# Autodesk Inventor assembly: Luftkissenboot
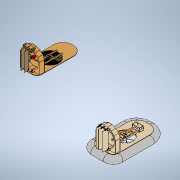
[picture p0: Inventor's stored thumbnail of the model, 180x180]
Saved by Autodesk Inventor 2020.3 (Build 243373010, 373A)
## iProperties
Company: HTBLuVA St. Pölten
Created: 2020-02-10
Part Number: Luftkissenboot
Document SubType Name: Assembly
Designer: Stefan Deimel
Mass: 445608 g
Surface Area: 116837 cm^2
Volume: 445608 cm^3
Density: 1 g/cm^3
Project: Diplomarbeit
Description: Luftkissenboot
Author: Stefan
Title: Luftkissenboot
Subject: Diplomarbeit
Revision Number: 3.1
## Documents named in this file (25)
- D:\Stefan\Schule\HTL\Diplomarbeit\git\Inventor\Luftkissenboot.iam
- D:\Stefan\Schule\HTL\Diplomarbeit\git\Inventor\Schlauchoot.ipt
- D:\Stefan\Schule\HTL\Diplomarbeit\git\Inventor\Aufbau.ipt
- D:\Stefan\Schule\HTL\Diplomarbeit\git\Inventor\Motor.ipt
- D:\Stefan\Schule\HTL\Diplomarbeit\git\Inventor\LenkungHinten.ipt
- D:\Stefan\Schule\HTL\Diplomarbeit\git\Inventor\Lenkung_hinten_verbindung.ipt
- D:\Stefan\Schule\HTL\Diplomarbeit\git\Inventor\Lenkung_vorne.ipt
- D:\Stefan\Schule\HTL\Diplomarbeit\git\Inventor\Propeller.ipt
- D:\Stefan\Schule\HTL\Diplomarbeit\git\Inventor\GitterUnten.ipt
- D:\Stefan\Schule\HTL\Diplomarbeit\git\Inventor\FahneHolz.ipt
- D:\Stefan\Schule\HTL\Diplomarbeit\git\Inventor\Fahnen_Halter v8.ipt
- D:\Stefan\Schule\HTL\Diplomarbeit\git\Inventor\Fahnen_Halter v8_1.ipt
- C:\Users\Stefan\Documents\Inventor\Content Center Files\R2020\de-DE\ANSI B18.2.4.2M\ANSI B18.2.4.2M - M5x0,8 - 8.ipt
- C:\Users\Stefan\Documents\Inventor\Content Center Files\R2020\de-DE\ISO 4016\ISO 4016 - M5 x 30.ipt
- D:\Stefan\Schule\HTL\Diplomarbeit\git\Inventor\FahenVerbindung_maybe.ipt
- D:\Stefan\Schule\HTL\Diplomarbeit\git\Inventor\Lenker\Lenkung.iam
- D:\Stefan\Schule\HTL\Diplomarbeit\git\Inventor\Servo.ipt
- D:\Stefan\Schule\HTL\Diplomarbeit\git\Inventor\HolzServoHalterMainPlatte1.ipt
- D:\Stefan\Schule\HTL\Diplomarbeit\git\Inventor\HalterungServosHochSeitlich.ipt
- D:\Stefan\Schule\HTL\Diplomarbeit\git\Inventor\HolzServoHalterHochLang.ipt
- D:\Stefan\Schule\HTL\Diplomarbeit\git\Inventor\HalterungServoHochSeitlich2.ipt
- D:\Stefan\Schule\HTL\Diplomarbeit\git\Inventor\Lenker\Skizzen\HolzServoHalterHinten.ipt
- D:\Stefan\Schule\HTL\Diplomarbeit\git\Inventor\Bodenplatte\Bodenplatte.iam
- C:\Users\Stefan\Documents\Inventor\Content Center Files\R2020\de-DE\ISO 4016\ISO 4016 - M6 x 30.ipt
- D:\Stefan\Schule\HTL\Diplomarbeit\git\Inventor\hintererAufbau\hintererAufbau.iam
## Components (121 placed, 24 different names)
1. Schlauchoot:1
2. Aufbau:1 — Starr:3, Starr:6, Drehbar:24, Drehbar:28, Drehbar:29, Drehbar:30, Drehbar:31, Drehbar:32, Starr:54
3. Motor:2 — Drehbar:27, Passend:3, Passend:4
4. LenkungHinten:2 — Drehbar:6
5. LenkungHinten:3 — Drehbar:7
6. Lenkung_hinten_verbindung:1 — Drehbar:6, Drehbar:7
7. Lenkung_vorne:1
8. Propeller:1 — Drehbar:26, Drehbar:27
9. Propeller:2 — Drehbar:26, Einfügen:11, Einfügen:12, Einfügen:13, Einfügen:14, Einfügen:15, Einfügen:16
10. GitterUnten:1 — Starr:3
11. Motor:3 — Drehbar:23, Starr:6
12. Propeller:5 — Drehbar:23, Einfügen:17, Einfügen:18, Einfügen:19, Einfügen:20, Einfügen:21, Einfügen:22
13. FahneHolz:1 — Starr:13, Starr:34, Starr:39
14. FahneHolz:2 — Starr:35, Starr:36, Starr:40
15. FahneHolz:3 — Starr:37, Starr:38, Starr:41
16. Fahnen_Halter v8:1 — Drehbar:24, Starr:7, Starr:13, Einfügen:60, Einfügen:61, Einfügen:62, Einfügen:63, Einfügen:64, Einfügen:65, Einfügen:66, Einfügen:67, Drehbar:38
17. Fahnen_Halter v8_1:1 — Einfügen:2, Starr:7
18. Fahnen_Halter v8:2 — Drehbar:29, Starr:9, Starr:37, Einfügen:40, Einfügen:41, Einfügen:42, Einfügen:43, Einfügen:72, Einfügen:73, Einfügen:74, Einfügen:75, Drehbar:37
19. Fahnen_Halter v8:3 — Drehbar:28, Starr:8, Starr:35, Einfügen:56, Einfügen:57, Einfügen:58, Einfügen:59, Einfügen:68, Einfügen:69, Einfügen:70, Einfügen:71, Drehbar:36
20. Fahnen_Halter v8:4 — Drehbar:32, Starr:12, Starr:38, Einfügen:52, Einfügen:53, Einfügen:54, Einfügen:55, Einfügen:76, Einfügen:77, Einfügen:78, Einfügen:79
21. Fahnen_Halter v8:5 — Drehbar:31, Starr:11, Starr:36, Einfügen:48, Einfügen:49, Einfügen:50, Einfügen:51, Einfügen:80, Einfügen:81, Einfügen:82, Einfügen:83
22. Fahnen_Halter v8:6 — Drehbar:30, Starr:10, Starr:34, Einfügen:44, Einfügen:45, Einfügen:46, Einfügen:47, Einfügen:84, Einfügen:85, Einfügen:86, Einfügen:87
23. Fahnen_Halter v8_1:2 — Starr:10, Einfügen:25, Einfügen:30
24. Fahnen_Halter v8_1:3 — Starr:11, Einfügen:26, Einfügen:31
25. Fahnen_Halter v8_1:4 — Starr:12, Einfügen:27, Passend:2
26. Fahnen_Halter v8_1:5 — Starr:8, Einfügen:23, Einfügen:28
27. Fahnen_Halter v8_1:6 — Starr:9, Einfügen:24, Einfügen:29
28. Fahnen_Halter v8:7 — Starr:39, Drehbar:34
29. Fahnen_Halter v8:8 — Starr:40, Drehbar:33
30. Fahnen_Halter v8:9 — Starr:41, Drehbar:35
31. FahenVerbindung_maybe:1 — Drehbar:33, Drehbar:34, Drehbar:35
32. Lenkung:1 [sub-assembly] — Passend:5, Passend:7
33. Servo:1 — Drehbar:36, Starr:46
34. Servo:2 — Drehbar:37, Starr:47
35. Servo:3 — Drehbar:38, Starr:48
36. HolzServoHalterHochLang:1 — Starr:50, Starr:53, Starr:54, Starr:55, Starr:56
37. HalterungServosHochSeitlich:4 — Starr:53
38. HalterungServoHochSeitlich2:1 — Starr:56
39. HalterungServoHochSeitlich2:2 — Starr:55, Starr:57
40. HolzServoHalterHinten:1 — Starr:57
41. Bodenplatte:1 [sub-assembly] — Passend:3, Einfügen:88, Einfügen:89, Einfügen:90, Einfügen:91, Passend:5, Passend:6, Passend:7
42. ISO 4016 M6 x 30:1 — Einfügen:88
43. ISO 4016 M6 x 30:2 — Einfügen:89
44. ISO 4016 M6 x 30:3 — Einfügen:90, Passend:4
45. ISO 4016 M6 x 30:4 — Einfügen:91
46. hintererAufbau:1 [sub-assembly] — Passend:6
47. ISO 4016 M5 x 30:1
48. ANSI B18.2.4.2M M5x0,8:1 — Einfügen:2
49. ISO 4016 M5 x 30:4 — Einfügen:11
50. ISO 4016 M5 x 30:5 — Einfügen:12
51. ISO 4016 M5 x 30:6 — Einfügen:13
52. ISO 4016 M5 x 30:7 — Einfügen:14
53. ISO 4016 M5 x 30:8 — Einfügen:15
54. ISO 4016 M5 x 30:9 — Einfügen:16
55. ISO 4016 M5 x 30:10 — Einfügen:17
56. ISO 4016 M5 x 30:11 — Einfügen:18
57. ISO 4016 M5 x 30:12 — Einfügen:19
58. ISO 4016 M5 x 30:13 — Einfügen:20
59. ISO 4016 M5 x 30:14 — Einfügen:21
60. ISO 4016 M5 x 30:15 — Einfügen:22
61. ISO 4016 M5 x 30:2 — Einfügen:23
62. ISO 4016 M5 x 30:3 — Einfügen:24
63. ISO 4016 M5 x 30:16 — Einfügen:25
64. ISO 4016 M5 x 30:17 — Einfügen:26
65. ISO 4016 M5 x 30:18 — Einfügen:27, Passend:1
66. ANSI B18.2.4.2M M5x0,8:2 — Einfügen:28
67. ANSI B18.2.4.2M M5x0,8:3 — Einfügen:29
68. ANSI B18.2.4.2M M5x0,8:4 — Einfügen:30
69. ANSI B18.2.4.2M M5x0,8:5 — Einfügen:31
70. ANSI B18.2.4.2M M5x0,8:6 — Passend:1, Passend:2
71. ISO 4016 M5 x 30:19 — Einfügen:40
72. ISO 4016 M5 x 30:20 — Einfügen:41
73. ISO 4016 M5 x 30:21 — Einfügen:42
74. ISO 4016 M5 x 30:22 — Einfügen:43
75. ISO 4016 M5 x 30:23 — Einfügen:44
76. ISO 4016 M5 x 30:24 — Einfügen:45
77. ISO 4016 M5 x 30:25 — Einfügen:46
78. ISO 4016 M5 x 30:26 — Einfügen:47
79. ISO 4016 M5 x 30:27 — Einfügen:48
80. ISO 4016 M5 x 30:28 — Einfügen:49
81. ISO 4016 M5 x 30:29 — Einfügen:50
82. ISO 4016 M5 x 30:30 — Einfügen:51
83. ISO 4016 M5 x 30:31 — Einfügen:52
84. ISO 4016 M5 x 30:32 — Einfügen:53
85. ISO 4016 M5 x 30:33 — Einfügen:54
86. ISO 4016 M5 x 30:34 — Einfügen:55
87. ISO 4016 M5 x 30:35 — Einfügen:56
88. ISO 4016 M5 x 30:36 — Einfügen:57
89. ISO 4016 M5 x 30:37 — Einfügen:58
90. ISO 4016 M5 x 30:38 — Einfügen:59
91. ISO 4016 M5 x 30:39 — Einfügen:60
92. ISO 4016 M5 x 30:40 — Einfügen:61
93. ISO 4016 M5 x 30:41 — Einfügen:62
94. ISO 4016 M5 x 30:42 — Einfügen:63
95. ANSI B18.2.4.2M M5x0,8:7 — Einfügen:64
96. ANSI B18.2.4.2M M5x0,8:8 — Einfügen:65
97. ANSI B18.2.4.2M M5x0,8:9 — Einfügen:66
98. ANSI B18.2.4.2M M5x0,8:10 — Einfügen:67
99. ANSI B18.2.4.2M M5x0,8:11 — Einfügen:68
100. ANSI B18.2.4.2M M5x0,8:12 — Einfügen:69
101. ANSI B18.2.4.2M M5x0,8:13 — Einfügen:70
102. ANSI B18.2.4.2M M5x0,8:14 — Einfügen:71
103. ANSI B18.2.4.2M M5x0,8:15 — Einfügen:72
104. ANSI B18.2.4.2M M5x0,8:16 — Einfügen:73
105. ANSI B18.2.4.2M M5x0,8:17 — Einfügen:74
106. ANSI B18.2.4.2M M5x0,8:18 — Einfügen:75
107. ANSI B18.2.4.2M M5x0,8:19 — Einfügen:76
108. ANSI B18.2.4.2M M5x0,8:20 — Einfügen:77
109. ANSI B18.2.4.2M M5x0,8:21 — Einfügen:78
110. ANSI B18.2.4.2M M5x0,8:22 — Einfügen:79
111. ANSI B18.2.4.2M M5x0,8:23 — Einfügen:80
112. ANSI B18.2.4.2M M5x0,8:24 — Einfügen:81
113. ANSI B18.2.4.2M M5x0,8:25 — Einfügen:82
114. ANSI B18.2.4.2M M5x0,8:26 — Einfügen:83
115. ANSI B18.2.4.2M M5x0,8:27 — Einfügen:84
116. ANSI B18.2.4.2M M5x0,8:28 — Einfügen:85
117. ANSI B18.2.4.2M M5x0,8:29 — Einfügen:86
118. ANSI B18.2.4.2M M5x0,8:30 — Einfügen:87
119. HalterungServosHochSeitlich:1 — Starr:50
120. HolzServoHalterMainPlatte1:1 — Starr:45, Starr:46, Starr:47, Starr:48
121. HolzServoHalterMainPlatte1:2 — Starr:45
## Relationships (126: Insert 75, WeldJoint 27, RevoluteJoint 17, Mate 7)
- Drehbar:6 [RevoluteJoint]: LenkungHinten:2 ↔ Lenkung_hinten_verbindung:1
- Drehbar:7 [RevoluteJoint]: LenkungHinten:3 ↔ Lenkung_hinten_verbindung:1
- Starr:3 [WeldJoint] (10 mm): Aufbau:1 ↔ GitterUnten:1
- Drehbar:23 [RevoluteJoint] (15 mm): Motor:3 ↔ Propeller:5
- Starr:6 [WeldJoint]: Aufbau:1 ↔ Motor:3
- Drehbar:24 [RevoluteJoint]: Aufbau:1 ↔ Fahnen_Halter v8:1
- [Insert]: Fahnen_Halter v8_1:1 ↔ ISO 4016 M5 x 30:1
- Einfügen:2 [Insert]: Fahnen_Halter v8_1:1 ↔ ANSI B18.2.4.2M M5x0,8:1
- Starr:7 [WeldJoint] (0.3 mm): Fahnen_Halter v8:1 ↔ Fahnen_Halter v8_1:1
- Drehbar:26 [RevoluteJoint]: Propeller:1 ↔ Propeller:2
- Drehbar:27 [RevoluteJoint]: Motor:2 ↔ Propeller:1
- Einfügen:11 [Insert]: Propeller:2 ↔ ISO 4016 M5 x 30:4
- Einfügen:12 [Insert]: Propeller:2 ↔ ISO 4016 M5 x 30:5
- Einfügen:13 [Insert]: Propeller:2 ↔ ISO 4016 M5 x 30:6
- Einfügen:14 [Insert]: Propeller:2 ↔ ISO 4016 M5 x 30:7
- Einfügen:15 [Insert]: Propeller:2 ↔ ISO 4016 M5 x 30:8
- Einfügen:16 [Insert]: Propeller:2 ↔ ISO 4016 M5 x 30:9
- Einfügen:17 [Insert]: Propeller:5 ↔ ISO 4016 M5 x 30:10
- Einfügen:18 [Insert]: Propeller:5 ↔ ISO 4016 M5 x 30:11
- Einfügen:19 [Insert]: Propeller:5 ↔ ISO 4016 M5 x 30:12
- Einfügen:20 [Insert]: Propeller:5 ↔ ISO 4016 M5 x 30:13
- Einfügen:21 [Insert]: Propeller:5 ↔ ISO 4016 M5 x 30:14
- Einfügen:22 [Insert]: Propeller:5 ↔ ISO 4016 M5 x 30:15
- Drehbar:28 [RevoluteJoint]: Aufbau:1 ↔ Fahnen_Halter v8:3
- Drehbar:29 [RevoluteJoint]: Aufbau:1 ↔ Fahnen_Halter v8:2
- Drehbar:30 [RevoluteJoint]: Aufbau:1 ↔ Fahnen_Halter v8:6
- Drehbar:31 [RevoluteJoint]: Aufbau:1 ↔ Fahnen_Halter v8:5
- Drehbar:32 [RevoluteJoint]: Aufbau:1 ↔ Fahnen_Halter v8:4
- Starr:8 [WeldJoint] (-0.3 mm): Fahnen_Halter v8:3 ↔ Fahnen_Halter v8_1:5
- Starr:9 [WeldJoint] (-0.3 mm): Fahnen_Halter v8:2 ↔ Fahnen_Halter v8_1:6
- Starr:10 [WeldJoint] (-0.3 mm): Fahnen_Halter v8:6 ↔ Fahnen_Halter v8_1:2
- Starr:11 [WeldJoint] (0.3 mm): Fahnen_Halter v8:5 ↔ Fahnen_Halter v8_1:3
- Starr:12 [WeldJoint] (-0.3 mm): Fahnen_Halter v8:4 ↔ Fahnen_Halter v8_1:4
- Einfügen:23 [Insert]: Fahnen_Halter v8_1:5 ↔ ISO 4016 M5 x 30:2
- Einfügen:24 [Insert]: Fahnen_Halter v8_1:6 ↔ ISO 4016 M5 x 30:3
- Einfügen:25 [Insert]: Fahnen_Halter v8_1:2 ↔ ISO 4016 M5 x 30:16
- Einfügen:26 [Insert]: Fahnen_Halter v8_1:3 ↔ ISO 4016 M5 x 30:17
- Einfügen:27 [Insert]: Fahnen_Halter v8_1:4 ↔ ISO 4016 M5 x 30:18
- Einfügen:28 [Insert]: Fahnen_Halter v8_1:5 ↔ ANSI B18.2.4.2M M5x0,8:2
- Einfügen:29 [Insert]: Fahnen_Halter v8_1:6 ↔ ANSI B18.2.4.2M M5x0,8:3
- Einfügen:30 [Insert]: Fahnen_Halter v8_1:2 ↔ ANSI B18.2.4.2M M5x0,8:4
- Einfügen:31 [Insert]: Fahnen_Halter v8_1:3 ↔ ANSI B18.2.4.2M M5x0,8:5
- Passend:1 [Mate]: ISO 4016 M5 x 30:18 ↔ ANSI B18.2.4.2M M5x0,8:6
- Passend:2 [Mate]: Fahnen_Halter v8_1:4 ↔ ANSI B18.2.4.2M M5x0,8:6
- Starr:13 [WeldJoint] (-0.1 mm): FahneHolz:1 ↔ Fahnen_Halter v8:1
- Starr:34 [WeldJoint] (-0.1 mm): FahneHolz:1 ↔ Fahnen_Halter v8:6
- Starr:35 [WeldJoint] (-0.1 mm): FahneHolz:2 ↔ Fahnen_Halter v8:3
- Starr:36 [WeldJoint] (-0.1 mm): FahneHolz:2 ↔ Fahnen_Halter v8:5
- Starr:37 [WeldJoint] (-0.1 mm): FahneHolz:3 ↔ Fahnen_Halter v8:2
- Starr:38 [WeldJoint] (-0.1 mm): FahneHolz:3 ↔ Fahnen_Halter v8:4
- Einfügen:40 [Insert]: Fahnen_Halter v8:2 ↔ ISO 4016 M5 x 30:19
- Einfügen:41 [Insert]: Fahnen_Halter v8:2 ↔ ISO 4016 M5 x 30:20
- Einfügen:42 [Insert]: Fahnen_Halter v8:2 ↔ ISO 4016 M5 x 30:21
- Einfügen:43 [Insert]: Fahnen_Halter v8:2 ↔ ISO 4016 M5 x 30:22
- Einfügen:44 [Insert]: Fahnen_Halter v8:6 ↔ ISO 4016 M5 x 30:23
- Einfügen:45 [Insert]: Fahnen_Halter v8:6 ↔ ISO 4016 M5 x 30:24
- Einfügen:46 [Insert]: Fahnen_Halter v8:6 ↔ ISO 4016 M5 x 30:25
- Einfügen:47 [Insert]: Fahnen_Halter v8:6 ↔ ISO 4016 M5 x 30:26
- Einfügen:48 [Insert]: Fahnen_Halter v8:5 ↔ ISO 4016 M5 x 30:27
- Einfügen:49 [Insert]: Fahnen_Halter v8:5 ↔ ISO 4016 M5 x 30:28
- Einfügen:50 [Insert]: Fahnen_Halter v8:5 ↔ ISO 4016 M5 x 30:29
- Einfügen:51 [Insert]: Fahnen_Halter v8:5 ↔ ISO 4016 M5 x 30:30
- Einfügen:52 [Insert]: Fahnen_Halter v8:4 ↔ ISO 4016 M5 x 30:31
- Einfügen:53 [Insert]: Fahnen_Halter v8:4 ↔ ISO 4016 M5 x 30:32
- Einfügen:54 [Insert]: Fahnen_Halter v8:4 ↔ ISO 4016 M5 x 30:33
- Einfügen:55 [Insert]: Fahnen_Halter v8:4 ↔ ISO 4016 M5 x 30:34
- Einfügen:56 [Insert]: Fahnen_Halter v8:3 ↔ ISO 4016 M5 x 30:35
- Einfügen:57 [Insert]: Fahnen_Halter v8:3 ↔ ISO 4016 M5 x 30:36
- Einfügen:58 [Insert]: Fahnen_Halter v8:3 ↔ ISO 4016 M5 x 30:37
- Einfügen:59 [Insert]: Fahnen_Halter v8:3 ↔ ISO 4016 M5 x 30:38
- Einfügen:60 [Insert]: Fahnen_Halter v8:1 ↔ ISO 4016 M5 x 30:39
- Einfügen:61 [Insert]: Fahnen_Halter v8:1 ↔ ISO 4016 M5 x 30:40
- Einfügen:62 [Insert]: Fahnen_Halter v8:1 ↔ ISO 4016 M5 x 30:41
- Einfügen:63 [Insert]: Fahnen_Halter v8:1 ↔ ISO 4016 M5 x 30:42
- Einfügen:64 [Insert]: Fahnen_Halter v8:1 ↔ ANSI B18.2.4.2M M5x0,8:7
- Einfügen:65 [Insert]: Fahnen_Halter v8:1 ↔ ANSI B18.2.4.2M M5x0,8:8
- Einfügen:66 [Insert]: Fahnen_Halter v8:1 ↔ ANSI B18.2.4.2M M5x0,8:9
- Einfügen:67 [Insert]: Fahnen_Halter v8:1 ↔ ANSI B18.2.4.2M M5x0,8:10
- Einfügen:68 [Insert]: Fahnen_Halter v8:3 ↔ ANSI B18.2.4.2M M5x0,8:11
- Einfügen:69 [Insert]: Fahnen_Halter v8:3 ↔ ANSI B18.2.4.2M M5x0,8:12
- Einfügen:70 [Insert]: Fahnen_Halter v8:3 ↔ ANSI B18.2.4.2M M5x0,8:13
- Einfügen:71 [Insert]: Fahnen_Halter v8:3 ↔ ANSI B18.2.4.2M M5x0,8:14
- Einfügen:72 [Insert]: Fahnen_Halter v8:2 ↔ ANSI B18.2.4.2M M5x0,8:15
- Einfügen:73 [Insert]: Fahnen_Halter v8:2 ↔ ANSI B18.2.4.2M M5x0,8:16
- Einfügen:74 [Insert]: Fahnen_Halter v8:2 ↔ ANSI B18.2.4.2M M5x0,8:17
- Einfügen:75 [Insert]: Fahnen_Halter v8:2 ↔ ANSI B18.2.4.2M M5x0,8:18
- Einfügen:76 [Insert]: Fahnen_Halter v8:4 ↔ ANSI B18.2.4.2M M5x0,8:19
- Einfügen:77 [Insert]: Fahnen_Halter v8:4 ↔ ANSI B18.2.4.2M M5x0,8:20
- Einfügen:78 [Insert]: Fahnen_Halter v8:4 ↔ ANSI B18.2.4.2M M5x0,8:21
- Einfügen:79 [Insert]: Fahnen_Halter v8:4 ↔ ANSI B18.2.4.2M M5x0,8:22
- Einfügen:80 [Insert]: Fahnen_Halter v8:5 ↔ ANSI B18.2.4.2M M5x0,8:23
- Einfügen:81 [Insert]: Fahnen_Halter v8:5 ↔ ANSI B18.2.4.2M M5x0,8:24
- Einfügen:82 [Insert]: Fahnen_Halter v8:5 ↔ ANSI B18.2.4.2M M5x0,8:25
- Einfügen:83 [Insert]: Fahnen_Halter v8:5 ↔ ANSI B18.2.4.2M M5x0,8:26
- Einfügen:84 [Insert]: Fahnen_Halter v8:6 ↔ ANSI B18.2.4.2M M5x0,8:27
- Einfügen:85 [Insert]: Fahnen_Halter v8:6 ↔ ANSI B18.2.4.2M M5x0,8:28
- Einfügen:86 [Insert]: Fahnen_Halter v8:6 ↔ ANSI B18.2.4.2M M5x0,8:29
- Einfügen:87 [Insert]: Fahnen_Halter v8:6 ↔ ANSI B18.2.4.2M M5x0,8:30
- Starr:39 [WeldJoint]: FahneHolz:1 ↔ Fahnen_Halter v8:7
- Starr:40 [WeldJoint]: FahneHolz:2 ↔ Fahnen_Halter v8:8
- Starr:41 [WeldJoint]: FahneHolz:3 ↔ Fahnen_Halter v8:9
- Drehbar:33 [RevoluteJoint]: Fahnen_Halter v8:8 ↔ FahenVerbindung_maybe:1
- Drehbar:34 [RevoluteJoint]: Fahnen_Halter v8:7 ↔ FahenVerbindung_maybe:1
- Drehbar:35 [RevoluteJoint]: Fahnen_Halter v8:9 ↔ FahenVerbindung_maybe:1
- Drehbar:36 [RevoluteJoint] (3.5 mm): Fahnen_Halter v8:3 ↔ Servo:1
- Drehbar:37 [RevoluteJoint] (3.5 mm): Fahnen_Halter v8:2 ↔ Servo:2
- Drehbar:38 [RevoluteJoint] (3.5 mm): Fahnen_Halter v8:1 ↔ Servo:3
- Starr:45 [WeldJoint]: HolzServoHalterMainPlatte1:1 ↔ HolzServoHalterMainPlatte1:2
- Starr:46 [WeldJoint]: Servo:1 ↔ HolzServoHalterMainPlatte1:1
- Starr:47 [WeldJoint]: Servo:2 ↔ HolzServoHalterMainPlatte1:1
- Starr:48 [WeldJoint]: Servo:3 ↔ HolzServoHalterMainPlatte1:1
- Starr:50 [WeldJoint]: HolzServoHalterHochLang:1 ↔ HalterungServosHochSeitlich:1
- Starr:53 [WeldJoint]: HolzServoHalterHochLang:1 ↔ HalterungServosHochSeitlich:4
- Starr:54 [WeldJoint]: Aufbau:1 ↔ HolzServoHalterHochLang:1
- Starr:55 [WeldJoint]: HolzServoHalterHochLang:1 ↔ HalterungServoHochSeitlich2:2
- Starr:56 [WeldJoint]: HolzServoHalterHochLang:1 ↔ HalterungServoHochSeitlich2:1
- Starr:57 [WeldJoint]: HalterungServoHochSeitlich2:2 ↔ HolzServoHalterHinten:1
- Passend:3 [Mate]: Motor:2 ↔ Bodenplatte:1
- Einfügen:88 [Insert]: Bodenplatte:1 ↔ ISO 4016 M6 x 30:1
- Einfügen:89 [Insert]: Bodenplatte:1 ↔ ISO 4016 M6 x 30:2
- Einfügen:90 [Insert]: Bodenplatte:1 ↔ ISO 4016 M6 x 30:3
- Einfügen:91 [Insert]: Bodenplatte:1 ↔ ISO 4016 M6 x 30:4
- Passend:4 [Mate]: Motor:2 ↔ ISO 4016 M6 x 30:3
- Passend:5 [Mate]: Lenkung:1 ↔ Bodenplatte:1
- Passend:6 [Mate]: Bodenplatte:1 ↔ hintererAufbau:1
- Passend:7 [Mate] (5 mm): Lenkung:1 ↔ Bodenplatte:1
